# Autodesk Inventor assembly: Undercarriage load and pannel
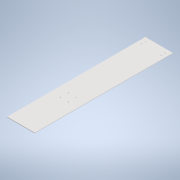
[picture p0: Inventor's stored thumbnail of the model, 180x180]
Saved by Autodesk Inventor 2020 (Build 240168000, 168)
## iProperties
Created: 2021-01-30
Part Number: Undercarriage load and pannel
Document SubType Name: Assembly
Designer: magda
Author: magda
## Documents named in this file (3)
- C:\Users\magda\OneDrive\Documents\Inventor\T3\Ramp Intake\Undercarriage load and pannel.iam
- C:\Users\magda\OneDrive\Documents\Inventor\T3\Ramp Intake\Undercarriage Panel.ipt
- C:\Users\magda\OneDrive\Documents\Inventor\T3\Ramp Intake\Undercarriage load.ipt
## Components (2 placed, 2 different names)
1. Undercarriage Panel:1 — Mate:1, Mate:2, Mate:3
2. Undercarriage load:1 — Mate:1, Mate:2, Mate:3
## Relationships (3: Mate 3)
- Mate:1: Undercarriage Panel:1 ↔ Undercarriage load:1
- Mate:2: Undercarriage Panel:1 ↔ Undercarriage load:1
- Mate:3: Undercarriage Panel:1 ↔ Undercarriage load:1
